(part 1 of 2)
# Autodesk Inventor assembly: gantry_assembly
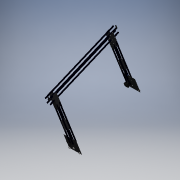
[picture p0: Inventor's stored thumbnail of the model, 180x180]
Saved by Autodesk Inventor 2018 (Build 220112000, 112)
## iProperties
Created: 2017-11-16
Part Number: gantry_assembly
Document SubType Name: Assembly
Designer: g
Author: g
## Documents named in this file (29)
- C:\Users\g\Desktop\AUG_inventor\gantry_assembly.iam
- C:\Users\g\Desktop\AUG_inventor\makerbeam600mm.ipt
- C:\Users\g\Desktop\AUG_inventor\tieplate_small.ipt
- C:\Users\g\Desktop\AUG_inventor\tieplate_big.ipt
- C:\Users\g\Desktop\AUG_inventor\M3 X 10mm Screw.ipt
- C:\Users\g\Desktop\AUG_inventor\M3_Lock_Nut(Thin_Nut).ipt
- C:\Users\g\Desktop\AUG_inventor\tieplate_small_MIR2.ipt
- C:\Users\g\Desktop\AUG_inventor\makerbeam876mm.ipt
- C:\Users\g\Desktop\AUG_inventor\makerbeam600mm_MIR.ipt
- C:\Users\g\Desktop\AUG_inventor\tieplate_small_MIR3.ipt
- C:\Users\g\Desktop\AUG_inventor\tieplate_big_MIR.ipt
- C:\Users\g\Desktop\AUG_inventor\M3 X 10mm Screw_MIR5.ipt
- C:\Users\g\Desktop\AUG_inventor\M3_Lock_Nut(Thin_Nut)_MIR8.ipt
- C:\Users\g\Desktop\AUG_inventor\tieplate_small_MIR2_MIR.ipt
- C:\Users\g\Desktop\AUG_inventor\NEMA17 w connector metric.ipt
- C:\Users\g\Desktop\AUG_inventor\GT2Pulley metric.ipt
- C:\Users\g\Desktop\AUG_inventor\GT2Bearing metric.ipt
- C:\Users\g\Desktop\AUG_inventor\M5 x 12mm Screw.ipt
- C:\Users\g\Desktop\AUG_inventor\M5 x 12mm Screw_MIR.ipt
- C:\Users\g\Desktop\AUG_inventor\m5x12mmscrew.ipt
- C:\Users\g\Desktop\AUG_inventor\5mmx20mmx8mm bearing.ipt
- C:\Users\g\Desktop\AUG_inventor\NEMA17 w connector metric_MIR.ipt
- C:\Users\g\Desktop\AUG_inventor\GT2Pulley metric_MIR.ipt
- C:\Users\g\Desktop\AUG_inventor\GT2Bearing metric_MIR.ipt
- C:\Users\g\Desktop\AUG_inventor\M5 x 12mm Screw_MIR1.ipt
- C:\Users\g\Desktop\AUG_inventor\M5 x 12mm Screw_MIR_MIR.ipt
- C:\Users\g\Desktop\AUG_inventor\m5x12mmscrew_MIR.ipt
- C:\Users\g\Desktop\AUG_inventor\5mmx20mmx8mm bearing_MIR.ipt
- C:\Users\g\Desktop\AUG_inventor\makerbeam_L-bracket.ipt
## Components (276 placed, 28 different names)
1. makerbeam600mm:1 — Mate:3, Flush:8, Flush:9, Mate:10, Flush:13, Flush:14, Mate:16, Slider:1, Slider:2, Flush:22, Slider:3, Flush:23, Slider:13, Slider:18, Slider:21, Slider:28, Slider:29, Slider:30, Flush:127, Flush:132, Flush:147, Flush:148
2. makerbeam600mm:2 — Mate:9, Flush:11, Mate:13, Flush:19, Flush:20, Mate:17, Mate:18, Flush:31, Flush:32, Mate:40, Slider:7, Flush:33, Slider:8, Slider:9, Flush:34, Slider:14, Slider:17, Slider:22, Slider:25, Slider:26, Slider:27, Slider:39, Slider:40, Mate:95, Flush:128, Flush:133, Flush:149, Flush:150
3. makerbeam600mm:3 — Mate:5, Flush:16, Mate:15, Flush:18, Flush:30, Mate:41, Slider:10, Slider:11, Slider:12, Slider:16, Slider:19, Slider:24, Slider:31, Slider:32, Slider:33, Slider:37, Slider:38, Mate:97, Flush:130, Flush:134, Flush:151, Flush:152
4. makerbeam600mm:4 — Flush:5, Flush:6, Mate:4, Mate:6, Flush:10, Mate:14, Flush:17, Flush:21, Slider:4, Slider:5, Slider:6, Flush:37, Slider:15, Slider:20, Slider:23, Slider:34, Slider:35, Slider:36, Flush:129, Flush:131
5. tieplate_small:2 — Mate:9, Mate:10, Mate:11, Flush:11, Flush:42, Flush:43, Flush:44, Flush:45, Flush:46, Flush:47, Mate:74, Mate:75, Mate:76, Mate:77, Mate:78, Mate:79
6. tieplate_small:3 — Mate:5, Mate:6, Mate:7, Flush:10, Flush:48, Flush:49, Flush:50, Flush:51, Flush:52, Flush:53, Mate:80, Mate:81, Mate:82, Mate:83, Mate:84, Mate:85
7. tieplate_small:5 — Flush:5, Flush:6, Mate:3, Flush:8, Flush:9, Mate:4, Mate:7, Mate:11, Mate:19, Mate:20, Mate:21, Mate:23, Mate:24, Mate:25, Mate:26, Mate:27, Mate:28, Mate:50, Mate:51, Flush:67, Flush:70, Flush:125, Flush:127, Flush:129, Flush:147, Symmetry:2
8. tieplate_small:6 — Mate:13, Flush:13, Flush:14, Mate:39, Mate:54, Mate:55, Mate:58, Mate:59, Mate:94, Mate:96, Flush:54, Flush:57, Flush:59, Flush:62, Mate:103, Mate:104, Mate:105, Flush:64, Flush:65, Mate:113, Mate:114, Flush:132, Flush:133, Flush:136, Flush:148, Flush:150
9. tieplate_small:7 — Mate:14, Flush:16, Mate:56, Mate:57, Mate:60, Mate:61, Mate:98, Mate:99, Flush:55, Flush:56, Flush:58, Flush:60, Mate:100, Mate:108, Mate:109, Flush:66, Mate:112, Mate:115, Mate:116, Mate:117, Flush:131, Flush:134, Flush:135, Flush:152
10. tieplate_small:8 — Mate:15, Flush:17, Flush:18, Mate:38, Mate:50, Mate:52, Flush:37, Flush:40, Flush:41, Mate:62, Mate:63, Mate:66, Mate:68, Mate:69, Mate:70, Flush:63, Mate:101, Mate:106, Mate:107, Flush:138
11. tieplate_small:9 — Mate:16, Flush:19, Flush:20, Mate:51, Mate:53, Flush:38, Flush:39, Mate:64, Mate:65, Mate:67, Mate:71, Mate:72, Mate:73, Flush:61, Mate:102, Mate:110, Mate:111, Flush:137
12. tieplate_big:1 — Mate:17, Mate:18, Flush:21, Mate:86, Mate:87, Mate:88, Mate:89, Mate:90, Mate:91, Mate:92, Mate:93, Mate:226, Flush:161, Flush:162, Mate:227, Flush:163, Mate:228, Flush:164, Mate:232, Mate:233, Mate:239, Mate:240, Mate:241, Mate:244, Cylindrical:107, Mate:245, Mate:246, Cylindrical:108, Cylindrical:109
13. M3 X 10mm Screw:1 — Cylindrical:9, Mate:44
14. M3 X 10mm Screw:2 — Cylindrical:10, Mate:45
15. M3 X 10mm Screw:3 — Cylindrical:11, Mate:48
16. M3 X 10mm Screw:4 — Cylindrical:2, Mate:25
17. M3 X 10mm Screw:5 — Cylindrical:1, Mate:24
18. M3 X 10mm Screw:6 — Cylindrical:5, Mate:26
19. M3 X 10mm Screw:7 — Cylindrical:6, Mate:27
20. M3 X 10mm Screw:8 — Cylindrical:7, Mate:47
21. M3 X 10mm Screw:9 — Cylindrical:16, Mate:60
22. M3 X 10mm Screw:10 — Cylindrical:17, Mate:59
23. M3 X 10mm Screw:11 — Cylindrical:15, Mate:61
24. M3 X 10mm Screw:12 — Cylindrical:14, Mate:49
25. M3 X 10mm Screw:13 — Cylindrical:4, Mate:23
26. M3 X 10mm Screw:14 — Cylindrical:3, Mate:28
27. M3 X 10mm Screw:15 — Cylindrical:8, Mate:46
28. M3_Lock_Nut(Thin_Nut):2 — Slider:20, Flush:41, Cylindrical:22
29. M3_Lock_Nut(Thin_Nut):3 — Slider:19, Flush:40, Cylindrical:21
30. M3_Lock_Nut(Thin_Nut):4 — Slider:18, Flush:39, Cylindrical:19
31. M3_Lock_Nut(Thin_Nut):5 — Slider:2, Flush:22, Cylindrical:2, Flush:25
32. M3_Lock_Nut(Thin_Nut):6 — Slider:1, Mate:19, Cylindrical:3, Flush:24
33. M3_Lock_Nut(Thin_Nut):7 — Slider:14, Mate:54, Cylindrical:18
34. M3_Lock_Nut(Thin_Nut):8 — Slider:17, Flush:38, Cylindrical:20
35. M3_Lock_Nut(Thin_Nut):9 — Slider:4, Flush:24, Cylindrical:6
36. M3_Lock_Nut(Thin_Nut):10 — Slider:5, Flush:25, Cylindrical:5
37. M3_Lock_Nut(Thin_Nut):11 — Slider:22, Mate:65, Cylindrical:23
38. M3_Lock_Nut(Thin_Nut):12 — Slider:13, Mate:55, Cylindrical:17
39. M3_Lock_Nut(Thin_Nut):13 — Slider:3, Flush:23, Cylindrical:1, Flush:26
40. M3_Lock_Nut(Thin_Nut):14 — Slider:6, Flush:26, Cylindrical:4
41. M3_Lock_Nut(Thin_Nut):15 — Slider:15, Mate:57, Cylindrical:15
42. M3_Lock_Nut(Thin_Nut):16 — Slider:16, Mate:56, Cylindrical:16
43. tieplate_small_MIR2:1 — Mate:36, Mate:37, Mate:38, Mate:39, Flush:30, Flush:31, Flush:32, Mate:40, Mate:41, Mate:42, Flush:35, Flush:36, Mate:43, Mate:44, Mate:45, Mate:46, Mate:47, Mate:48, Mate:49, Mate:52, Mate:53, Flush:68, Flush:69, Flush:126, Flush:128, Flush:130, Flush:149, Flush:151
44. M3_Lock_Nut(Thin_Nut):17 — Slider:10, Flush:35, Cylindrical:10
45. M3_Lock_Nut(Thin_Nut):18 — Slider:9, Flush:34, Cylindrical:8
46. M3_Lock_Nut(Thin_Nut):19 — Slider:12, Mate:43, Cylindrical:11
47. M3_Lock_Nut(Thin_Nut):20 — Slider:11, Flush:36, Cylindrical:14
48. M3_Lock_Nut(Thin_Nut):21 — Slider:8, Mate:42, Cylindrical:7
49. M3_Lock_Nut(Thin_Nut):22 — Slider:7, Flush:33, Cylindrical:9
50. M3 X 10mm Screw:16 — Cylindrical:18, Mate:58
51. M3_Lock_Nut(Thin_Nut):23 — Slider:24, Mate:62, Cylindrical:26
52. M3_Lock_Nut(Thin_Nut):24 — Slider:23, Mate:63, Cylindrical:25
53. M3_Lock_Nut(Thin_Nut):25 — Slider:21, Mate:64, Cylindrical:24
54. M3 X 10mm Screw:17 — Cylindrical:19, Mate:72
55. M3 X 10mm Screw:18 — Cylindrical:20, Mate:73
56. M3 X 10mm Screw:19 — Cylindrical:21, Mate:68
57. M3 X 10mm Screw:20 — Cylindrical:22, Mate:70
58. M3 X 10mm Screw:21 — Cylindrical:26, Mate:66
59. M3 X 10mm Screw:22 — Cylindrical:25, Mate:69
60. M3 X 10mm Screw:23 — Cylindrical:24, Mate:71
61. M3 X 10mm Screw:24 — Cylindrical:23, Mate:67
62. M3 X 10mm Screw:25 — Cylindrical:33, Mate:74
63. M3 X 10mm Screw:26 — Cylindrical:37, Mate:79
64. M3 X 10mm Screw:27 — Cylindrical:31, Mate:82
65. M3 X 10mm Screw:28 — Cylindrical:34, Mate:75
66. M3 X 10mm Screw:29 — Cylindrical:36, Mate:78
67. M3 X 10mm Screw:30 — Cylindrical:29, Mate:81
68. M3 X 10mm Screw:31 — Cylindrical:38, Mate:77
69. M3 X 10mm Screw:32 — Cylindrical:32, Mate:85
70. M3 X 10mm Screw:33 — Cylindrical:28, Mate:83
71. M3 X 10mm Screw:34 — Cylindrical:35, Mate:76
72. M3 X 10mm Screw:35 — Cylindrical:30, Mate:80
73. M3 X 10mm Screw:36 — Cylindrical:27, Mate:84
74. M3_Lock_Nut(Thin_Nut):26 — Slider:25, Flush:42, Cylindrical:37
75. M3_Lock_Nut(Thin_Nut):27 — Slider:26, Flush:44, Cylindrical:38
76. M3_Lock_Nut(Thin_Nut):28 — Slider:28, Flush:46, Cylindrical:34
77. M3_Lock_Nut(Thin_Nut):29 — Slider:27, Flush:43, Cylindrical:36
78. M3_Lock_Nut(Thin_Nut):30 — Slider:34, Flush:50, Cylindrical:27
79. M3_Lock_Nut(Thin_Nut):31 — Slider:32, Flush:53, Cylindrical:32
80. M3_Lock_Nut(Thin_Nut):32 — Slider:29, Flush:45, Cylindrical:33
81. M3_Lock_Nut(Thin_Nut):33 — Slider:33, Flush:51, Cylindrical:30
82. M3_Lock_Nut(Thin_Nut):34 — Slider:36, Flush:49, Cylindrical:28
83. M3_Lock_Nut(Thin_Nut):35 — Slider:30, Flush:47, Cylindrical:35
84. M3_Lock_Nut(Thin_Nut):36 — Slider:31, Flush:52, Cylindrical:31
85. M3_Lock_Nut(Thin_Nut):37 — Slider:35, Flush:48, Cylindrical:29
86. M3_Lock_Nut(Thin_Nut):39 — Slider:37, Mate:86, Cylindrical:42
87. M3_Lock_Nut(Thin_Nut):40 — Slider:38, Mate:87, Cylindrical:39
88. M3_Lock_Nut(Thin_Nut):41 — Slider:40, Mate:88, Cylindrical:41
89. M3_Lock_Nut(Thin_Nut):42 — Slider:39, Mate:89, Cylindrical:40
90. M3 X 10mm Screw:37 — Cylindrical:39, Mate:91
91. M3 X 10mm Screw:38 — Cylindrical:42, Mate:90
92. M3 X 10mm Screw:39 — Cylindrical:40, Mate:92
93. M3 X 10mm Screw:40 — Cylindrical:41, Mate:93
94. makerbeam876mm:1 — Mate:96, Flush:54, Flush:57, Slider:51, Slider:52, Flush:136, Flush:140, Slider:95, Slider:101, Flush:189, Flush:190, Flush:192
95. makerbeam876mm:2 — Mate:94, Mate:95, Flush:59, Slider:43, Slider:44, Slider:45, Slider:46, Flush:69, Flush:70, Flush:125, Flush:126, Flush:137, Flush:141, Slider:93, Slider:94, Slider:104, Slider:105, Flush:188, Flush:189
96. makerbeam876mm:3 — Mate:99, Flush:55, Flush:56, Slider:49, Slider:50, Symmetry:1, Flush:135, Flush:139, Slider:99, Slider:100, Flush:182, Mate:320, Flush:183, Flush:184, Flush:185, Mate:321, Slider:106, Slider:107, Flush:186, Slider:108, Slider:109, Flush:190, Flush:191
97. makerbeam876mm:4 — Mate:97, Mate:98, Flush:58, Slider:41, Slider:42, Slider:47, Slider:48, Flush:67, Flush:68, Symmetry:1, Flush:123, Flush:124, Flush:138, Flush:142, Slider:97, Slider:98, Slider:102, Slider:103, Flush:160, Flush:188, Flush:191, Flush:192
98. M3_Lock_Nut(Thin_Nut):43 — Slider:43, Mate:103, Cylindrical:49
99. M3_Lock_Nut(Thin_Nut):44 — Slider:42, Mate:101, Cylindrical:47
100. M3_Lock_Nut(Thin_Nut):45 — Slider:41, Flush:63, Cylindrical:48
101. M3_Lock_Nut(Thin_Nut):46 — Slider:44, Flush:62, Cylindrical:50
102. M3_Lock_Nut(Thin_Nut):47 — Slider:45, Flush:61, Cylindrical:45
103. M3_Lock_Nut(Thin_Nut):48 — Slider:46, Mate:102, Cylindrical:46
104. M3_Lock_Nut(Thin_Nut):49 — Slider:47, Flush:60, Cylindrical:44
105. M3_Lock_Nut(Thin_Nut):50 — Slider:48, Mate:100, Cylindrical:43
106. M3_Lock_Nut(Thin_Nut):51 — Slider:50, Flush:66, Cylindrical:51
107. M3_Lock_Nut(Thin_Nut):52 — Slider:52, Flush:65, Cylindrical:54
108. M3_Lock_Nut(Thin_Nut):53 — Slider:49, Mate:112, Cylindrical:52
109. M3_Lock_Nut(Thin_Nut):54 — Slider:51, Flush:64, Cylindrical:53
110. M3 X 10mm Screw:41 — Cylindrical:49, Mate:104
111. M3 X 10mm Screw:42 — Cylindrical:48, Mate:107
112. M3 X 10mm Screw:43 — Cylindrical:50, Mate:105
113. M3 X 10mm Screw:44 — Cylindrical:47, Mate:106
114. M3 X 10mm Screw:45 — Cylindrical:53, Mate:114
115. M3 X 10mm Screw:46 — Cylindrical:51, Mate:115
116. M3 X 10mm Screw:47 — Cylindrical:54, Mate:113
117. M3 X 10mm Screw:48 — Cylindrical:52, Mate:117
118. M3 X 10mm Screw:49 — Cylindrical:46, Mate:110
119. M3 X 10mm Screw:50 — Cylindrical:43, Mate:109, Mate:116
120. M3 X 10mm Screw:51 — Cylindrical:44, Mate:108
121. M3 X 10mm Screw:52 — Cylindrical:45, Mate:111
122. makerbeam600mm_MIR:1 — Mate:118, Flush:75, Flush:76, Mate:125, Flush:79, Flush:80, Mate:131, Flush:91, Flush:95, Slider:55, Slider:56, Slider:57, Slider:63, Slider:64, Slider:76, Slider:79, Slider:83, Slider:86
123. makerbeam600mm_MIR:2 — Flush:73, Mate:119, Mate:126, Flush:85, Flush:86, Mate:132, Mate:133, Mate:160, Flush:97, Flush:98, Flush:101, Flush:103, Slider:58, Slider:59, Slider:62, Slider:69, Slider:72, Slider:73, Slider:77, Slider:78, Slider:80, Slider:91, Slider:92
124. makerbeam600mm_MIR:3 — Mate:121, Flush:81, Flush:83, Mate:129, Mate:159, Flush:99, Slider:54, Slider:67, Slider:68, Slider:70, Slider:71, Slider:74, Slider:82, Slider:84, Slider:87, Slider:89, Slider:90, Flush:145, Flush:146
125. makerbeam600mm_MIR:4 — Flush:74, Mate:120, Mate:124, Flush:77, Flush:78, Mate:127, Flush:82, Flush:84, Flush:87, Slider:53, Slider:60, Slider:61, Slider:65, Slider:66, Slider:75, Slider:81, Slider:85, Slider:88, Flush:143, Flush:144
126. tieplate_small_MIR3:1 — Flush:73, Mate:118, Mate:119, Mate:122, Mate:179, Mate:180, Mate:182, Mate:183, Mate:185, Mate:188, Flush:104, Flush:105, Flush:106, Flush:107, Flush:110, Flush:113
127. tieplate_small_MIR3:2 — Flush:74, Mate:120, Mate:121, Mate:123, Mate:181, Mate:184, Mate:186, Mate:187, Mate:189, Mate:190, Flush:108, Flush:109, Flush:111, Flush:112, Flush:114, Flush:115
128. tieplate_small_MIR3:3 — Mate:122, Mate:123, Mate:124, Flush:75, Flush:76, Mate:125, Flush:77, Flush:78, Mate:128, Mate:130, Mate:134, Mate:135, Mate:136, Mate:137, Mate:141, Mate:142, Mate:143, Mate:149, Mate:150, Flush:123, Flush:143, Symmetry:2
129. tieplate_small_MIR3:4 — Flush:79, Flush:80, Mate:126, Mate:139, Mate:144, Mate:146, Mate:161, Mate:167, Mate:199, Flush:117, Flush:121, Mate:204, Mate:206, Mate:210, Flush:140, Flush:155, Mate:218, Mate:219, Mate:224, Mate:225
130. tieplate_small_MIR3:5 — Flush:81, Mate:127, Mate:138, Mate:140, Mate:147, Mate:148, Flush:119, Mate:202, Mate:209, Mate:211, Mate:213, Mate:214, Mate:215, Flush:139, Flush:144, Flush:146, Flush:153, Mate:217, Flush:154, Mate:220, Mate:221, Mate:222, Mate:223, Flush:160
131. tieplate_small_MIR3:6 — Flush:82, Mate:128, Flush:83, Flush:84, Mate:129, Flush:88, Flush:89, Mate:152, Mate:162, Mate:168, Mate:169, Mate:173, Mate:174, Mate:175, Mate:176, Mate:200, Flush:116, Mate:205, Mate:207, Flush:142
132. tieplate_small_MIR3:7 — Mate:130, Flush:85, Flush:86, Mate:131, Flush:90, Flush:92, Mate:145, Mate:151, Mate:170, Mate:171, Mate:172, Mate:177, Mate:178, Flush:118, Mate:201, Mate:212, Mate:216, Flush:141
133. tieplate_big_MIR:1 — Flush:87, Mate:132, Mate:133, Mate:191, Mate:192, Mate:193, Mate:194, Mate:195, Mate:196, Mate:197, Mate:198, Mate:250, Mate:251, Mate:252, Mate:253, Mate:255, Mate:256, Cylindrical:110, Cylindrical:111, Cylindrical:112, Mate:257, Flush:165, Mate:258, Mate:259, Mate:302, Mate:303, Mate:304
134. M3 X 10mm Screw_MIR5:1 — Mate:158, Cylindrical:69
135. M3 X 10mm Screw_MIR5:2 — Mate:157, Cylindrical:64
136. M3 X 10mm Screw_MIR5:3 — Mate:154, Cylindrical:66
137. M3 X 10mm Screw_MIR5:4 — Mate:134, Cylindrical:55
138. M3 X 10mm Screw_MIR5:5 — Mate:135, Cylindrical:60
139. M3 X 10mm Screw_MIR5:6 — Mate:136, Cylindrical:58
140. M3 X 10mm Screw_MIR5:7 — Mate:137, Cylindrical:57
141. M3 X 10mm Screw_MIR5:8 — Mate:155, Cylindrical:68
142. M3 X 10mm Screw_MIR5:9 — Mate:138, Cylindrical:63
143. M3 X 10mm Screw_MIR5:10 — Mate:139, Cylindrical:59
144. M3 X 10mm Screw_MIR5:11 — Mate:140, Cylindrical:62
145. M3 X 10mm Screw_MIR5:12 — Mate:153, Cylindrical:67
146. M3 X 10mm Screw_MIR5:13 — Mate:141, Cylindrical:61
147. M3 X 10mm Screw_MIR5:14 — Mate:142, Cylindrical:56
148. M3 X 10mm Screw_MIR5:15 — Mate:156, Cylindrical:65
149. M3_Lock_Nut(Thin_Nut)_MIR8:1 — Flush:88, Slider:53, Cylindrical:74
150. M3_Lock_Nut(Thin_Nut)_MIR8:2 — Flush:89, Slider:54, Cylindrical:73
151. M3_Lock_Nut(Thin_Nut)_MIR8:3 — Flush:90, Slider:55, Cylindrical:71
152. M3_Lock_Nut(Thin_Nut)_MIR8:4 — Flush:91, Flush:94, Cylindrical:55, Slider:56
153. M3_Lock_Nut(Thin_Nut)_MIR8:5 — Mate:143, Flush:93, Cylindrical:56, Slider:57
154. M3_Lock_Nut(Thin_Nut)_MIR8:6 — Mate:144, Slider:58, Cylindrical:70
155. M3_Lock_Nut(Thin_Nut)_MIR8:7 — Flush:92, Slider:59, Cylindrical:72
156. M3_Lock_Nut(Thin_Nut)_MIR8:8 — Flush:93, Cylindrical:57, Slider:60
157. M3_Lock_Nut(Thin_Nut)_MIR8:9 — Flush:94, Cylindrical:58, Slider:61
158. M3_Lock_Nut(Thin_Nut)_MIR8:10 — Mate:145, Slider:62, Cylindrical:78
159. M3_Lock_Nut(Thin_Nut)_MIR8:11 — Mate:146, Cylindrical:59, Slider:63
160. M3_Lock_Nut(Thin_Nut)_MIR8:12 — Flush:95, Flush:96, Cylindrical:60, Slider:64
161. M3_Lock_Nut(Thin_Nut)_MIR8:13 — Flush:96, Cylindrical:61, Slider:65
162. M3_Lock_Nut(Thin_Nut)_MIR8:14 — Mate:147, Cylindrical:62, Slider:66
163. M3_Lock_Nut(Thin_Nut)_MIR8:15 — Mate:148, Cylindrical:63, Slider:67
164. tieplate_small_MIR2_MIR:1 — Mate:151, Mate:152, Mate:153, Mate:154, Mate:155, Mate:156, Mate:157, Mate:158, Mate:159, Mate:160, Flush:97, Flush:98, Flush:99, Mate:161, Mate:162, Mate:163, Mate:164, Flush:100, Mate:165, Flush:102, Mate:166, Flush:124, Flush:145
165. M3_Lock_Nut(Thin_Nut)_MIR8:16 — Flush:100, Cylindrical:64, Slider:68
166. M3_Lock_Nut(Thin_Nut)_MIR8:17 — Flush:101, Cylindrical:65, Slider:69
167. M3_Lock_Nut(Thin_Nut)_MIR8:18 — Mate:165, Cylindrical:66, Slider:70
168. M3_Lock_Nut(Thin_Nut)_MIR8:19 — Flush:102, Cylindrical:67, Slider:71
169. M3_Lock_Nut(Thin_Nut)_MIR8:20 — Mate:166, Cylindrical:68, Slider:72
170. M3_Lock_Nut(Thin_Nut)_MIR8:21 — Flush:103, Cylindrical:69, Slider:73
171. M3 X 10mm Screw_MIR5:16 — Mate:167, Cylindrical:70
172. M3_Lock_Nut(Thin_Nut)_MIR8:22 — Mate:168, Slider:74, Cylindrical:75
173. M3_Lock_Nut(Thin_Nut)_MIR8:23 — Mate:169, Slider:75, Cylindrical:76
174. M3_Lock_Nut(Thin_Nut)_MIR8:24 — Mate:170, Slider:76, Cylindrical:77
175. M3 X 10mm Screw_MIR5:17 — Mate:171, Cylindrical:71
176. M3 X 10mm Screw_MIR5:18 — Mate:172, Cylindrical:72
177. M3 X 10mm Screw_MIR5:19 — Mate:173, Cylindrical:73
178. M3 X 10mm Screw_MIR5:20 — Mate:174, Cylindrical:74
179. M3 X 10mm Screw_MIR5:21 — Mate:175, Cylindrical:75
180. M3 X 10mm Screw_MIR5:22 — Mate:176, Cylindrical:76
181. M3 X 10mm Screw_MIR5:23 — Mate:177, Cylindrical:77
182. M3 X 10mm Screw_MIR5:24 — Mate:178, Cylindrical:78
183. M3 X 10mm Screw_MIR5:25 — Mate:179, Cylindrical:85
184. M3 X 10mm Screw_MIR5:26 — Mate:180, Cylindrical:79
185. M3 X 10mm Screw_MIR5:27 — Mate:181, Cylindrical:89
186. M3 X 10mm Screw_MIR5:28 — Mate:182, Cylindrical:81
187. M3 X 10mm Screw_MIR5:29 — Mate:183, Cylindrical:82
188. M3 X 10mm Screw_MIR5:30 — Mate:184, Cylindrical:90
189. M3 X 10mm Screw_MIR5:31 — Mate:185, Cylindrical:80
190. M3 X 10mm Screw_MIR5:32 — Mate:186, Cylindrical:84
191. M3 X 10mm Screw_MIR5:33 — Mate:187, Cylindrical:87
192. M3 X 10mm Screw_MIR5:34 — Mate:188, Cylindrical:88
193. M3 X 10mm Screw_MIR5:35 — Mate:189, Cylindrical:86
194. M3 X 10mm Screw_MIR5:36 — Mate:190, Cylindrical:83
195. M3_Lock_Nut(Thin_Nut)_MIR8:25 — Flush:104, Cylindrical:79, Slider:77
196. M3_Lock_Nut(Thin_Nut)_MIR8:26 — Flush:105, Cylindrical:80, Slider:78
197. M3_Lock_Nut(Thin_Nut)_MIR8:27 — Flush:106, Cylindrical:81, Slider:79
198. M3_Lock_Nut(Thin_Nut)_MIR8:28 — Flush:107, Cylindrical:82, Slider:80
199. M3_Lock_Nut(Thin_Nut)_MIR8:29 — Flush:108, Cylindrical:83, Slider:81
200. M3_Lock_Nut(Thin_Nut)_MIR8:30 — Flush:109, Cylindrical:84, Slider:82
201. M3_Lock_Nut(Thin_Nut)_MIR8:31 — Flush:110, Cylindrical:85, Slider:83
202. M3_Lock_Nut(Thin_Nut)_MIR8:32 — Flush:111, Cylindrical:86, Slider:84
203. M3_Lock_Nut(Thin_Nut)_MIR8:33 — Flush:112, Cylindrical:87, Slider:85
204. M3_Lock_Nut(Thin_Nut)_MIR8:34 — Flush:113, Cylindrical:88, Slider:86
205. M3_Lock_Nut(Thin_Nut)_MIR8:35 — Flush:114, Cylindrical:89, Slider:87
206. M3_Lock_Nut(Thin_Nut)_MIR8:36 — Flush:115, Cylindrical:90, Slider:88
207. M3_Lock_Nut(Thin_Nut)_MIR8:37 — Mate:191, Slider:89, Cylindrical:92
208. M3_Lock_Nut(Thin_Nut)_MIR8:38 — Mate:192, Slider:90, Cylindrical:91
209. M3_Lock_Nut(Thin_Nut)_MIR8:39 — Mate:193, Slider:91, Cylindrical:94
210. M3_Lock_Nut(Thin_Nut)_MIR8:40 — Mate:194, Slider:92, Cylindrical:93
211. M3 X 10mm Screw_MIR5:37 — Mate:195, Cylindrical:91
212. M3 X 10mm Screw_MIR5:38 — Mate:196, Cylindrical:92
213. M3 X 10mm Screw_MIR5:39 — Mate:197, Cylindrical:93
214. M3 X 10mm Screw_MIR5:40 — Mate:198, Cylindrical:94
215. M3_Lock_Nut(Thin_Nut)_MIR8:41 — Mate:199, Cylindrical:95, Slider:94
216. M3_Lock_Nut(Thin_Nut)_MIR8:42 — Mate:200, Cylindrical:98, Slider:103
217. M3_Lock_Nut(Thin_Nut)_MIR8:43 — Flush:116, Cylindrical:96, Slider:102
218. M3_Lock_Nut(Thin_Nut)_MIR8:44 — Flush:117, Cylindrical:97, Slider:93
219. M3_Lock_Nut(Thin_Nut)_MIR8:45 — Flush:118, Cylindrical:106, Slider:105
220. M3_Lock_Nut(Thin_Nut)_MIR8:46 — Mate:201, Cylindrical:103, Slider:104
221. M3_Lock_Nut(Thin_Nut)_MIR8:47 — Flush:119, Cylindrical:105, Slider:97, Flush:154
222. M3_Lock_Nut(Thin_Nut)_MIR8:48 — Mate:202, Cylindrical:104, Slider:98
223. M3_Lock_Nut(Thin_Nut)_MIR8:49 — Cylindrical:100, Slider:99, Mate:217
224. M3_Lock_Nut(Thin_Nut)_MIR8:50 — Flush:121, Cylindrical:101, Slider:95
225. M3_Lock_Nut(Thin_Nut)_MIR8:51 — Cylindrical:102, Slider:100, Flush:153
226. M3_Lock_Nut(Thin_Nut)_MIR8:52 — Cylindrical:99, Slider:101, Flush:155
227. M3 X 10mm Screw_MIR5:41 — Mate:204, Cylindrical:95, Mate:224
228. M3 X 10mm Screw_MIR5:42 — Mate:205, Cylindrical:96
229. M3 X 10mm Screw_MIR5:43 — Mate:206, Cylindrical:97, Mate:225
230. M3 X 10mm Screw_MIR5:44 — Mate:207, Cylindrical:98
231. M3 X 10mm Screw_MIR5:45 — Cylindrical:99, Mate:218
232. M3 X 10mm Screw_MIR5:46 — Mate:209, Cylindrical:100, Mate:221
233. M3 X 10mm Screw_MIR5:47 — Mate:210, Cylindrical:101, Mate:219
234. M3 X 10mm Screw_MIR5:48 — Mate:211, Cylindrical:102, Mate:220
235. M3 X 10mm Screw_MIR5:49 — Mate:212, Cylindrical:103
236. M3 X 10mm Screw_MIR5:50 — Mate:213, Mate:214, Cylindrical:104, Mate:223
237. M3 X 10mm Screw_MIR5:51 — Mate:215, Cylindrical:105, Mate:222
238. M3 X 10mm Screw_MIR5:52 — Mate:216, Cylindrical:106
239. NEMA17 w connector metric:3 — Mate:226, Flush:161, Flush:162, Mate:229, Mate:230, Mate:231, Rigid:3
240. GT2Pulley metric:1 — Rigid:3
241. GT2Bearing metric:3 — Rigid:4
242. GT2Bearing metric:4 — Rigid:2
243. M5 x 12mm Screw:1 — Mate:227, Flush:163, Mate:228, Rigid:2
244. M5 x 12mm Screw_MIR:1 — Flush:164, Mate:232, Mate:233, Rigid:4
245. m5x12mmscrew:1 — Mate:244, Cylindrical:107, Rotational:2
246. m5x12mmscrew:2 — Mate:245, Cylindrical:109, Rotational:1
247. m5x12mmscrew:3 — Mate:246, Cylindrical:108, Rotational:3
248. 5mmx20mmx8mm bearing:1 — Rotational:1
249. 5mmx20mmx8mm bearing:2 — Rotational:2
250. 5mmx20mmx8mm bearing:3 — Rotational:3
251. NEMA17 w connector metric_MIR:1 — Mate:247, Mate:248, Mate:249, Rigid:5, Mate:252, Mate:257, Flush:165
252. GT2Pulley metric_MIR:1 — Rigid:5
253. GT2Bearing metric_MIR:1 — Rigid:7
254. GT2Bearing metric_MIR:2 — Rigid:6
255. M5 x 12mm Screw_MIR1:1 — Rigid:6, Mate:253, Flush:166, Mate:303, Mate:304
256. M5 x 12mm Screw_MIR_MIR:1 — Rigid:7, Mate:258, Mate:259, Flush:166, Mate:302
257. m5x12mmscrew_MIR:1 — Rotational:5, Mate:251, Mate:256, Cylindrical:112
258. m5x12mmscrew_MIR:2 — Rotational:4, Mate:250, Cylindrical:110
259. m5x12mmscrew_MIR:3 — Rotational:6, Mate:255, Cylindrical:111
260. 5mmx20mmx8mm bearing_MIR:1 — Rotational:4
261. 5mmx20mmx8mm bearing_MIR:2 — Rotational:5
262. 5mmx20mmx8mm bearing_MIR:3 — Rotational:6
263. makerbeam_L-bracket:1 — Flush:182, Mate:320, Flush:183, Flush:187, Mate:323, Mate:325, Mate:326, Cylindrical:137, Mate:328, Mate:330
264. makerbeam_L-bracket:2 — Flush:184, Flush:185, Mate:321, Mate:322, Mate:324, Mate:327, Cylindrical:136, Mate:329, Mate:331
265. M3_Lock_Nut(Thin_Nut):55 — Slider:106, Mate:322, Cylindrical:135
266. M3_Lock_Nut(Thin_Nut):56 — Slider:107, Flush:186, Cylindrical:134
267. M3_Lock_Nut(Thin_Nut):57 — Slider:108, Mate:323, Cylindrical:132
268. M3_Lock_Nut(Thin_Nut):58 — Slider:109, Flush:187, Cylindrical:133
269. M3 X 10mm Screw:61 — Cylindrical:132, Mate:325
270. M3 X 10mm Screw:62 — Cylindrical:133, Mate:326
271. M3 X 10mm Screw:63 — Cylindrical:134, Mate:324
272. M3 X 10mm Screw:64 — Cylindrical:135, Mate:327
273. M3 X 10mm Screw:65 — Cylindrical:136, Mate:329, Cylindrical:138
274. M3 X 10mm Screw:66 — Cylindrical:137, Mate:328, Cylindrical:139
275. M3_Lock_Nut(Thin_Nut):59 — Cylindrical:138, Mate:331
276. M3_Lock_Nut(Thin_Nut):60 — Cylindrical:139, Mate:330
## Relationships (651: Mate 252, Flush 159, CylindricalJoint 118, TranslationJoint 108, WeldJoint 6, RevoluteJoint 6, Symmetry 2)
- Flush:5: makerbeam600mm:4 ↔ tieplate_small:5
- Flush:6: makerbeam600mm:4 ↔ tieplate_small:5
- Mate:3: makerbeam600mm:1 ↔ tieplate_small:5
- Flush:8: makerbeam600mm:1 ↔ tieplate_small:5
- Flush:9: makerbeam600mm:1 ↔ tieplate_small:5
- Mate:4: makerbeam600mm:4 ↔ tieplate_small:5
- Mate:5: makerbeam600mm:3 ↔ tieplate_small:3
- Mate:6: makerbeam600mm:4 ↔ tieplate_small:3
- Mate:7: tieplate_small:3 ↔ tieplate_small:5
- Flush:10 (300 mm): makerbeam600mm:4 ↔ tieplate_small:3
- Mate:9: makerbeam600mm:2 ↔ tieplate_small:2
- Mate:10: makerbeam600mm:1 ↔ tieplate_small:2
- Mate:11: tieplate_small:2 ↔ tieplate_small:5
- Flush:11 (300 mm): makerbeam600mm:2 ↔ tieplate_small:2
- Mate:13: makerbeam600mm:2 ↔ tieplate_small:6
- Flush:13: makerbeam600mm:1 ↔ tieplate_small:6
- Flush:14 (-72.5 mm): makerbeam600mm:1 ↔ tieplate_small:6
- Mate:14: makerbeam600mm:4 ↔ tieplate_small:7
- Flush:16 (-72.5 mm): makerbeam600mm:3 ↔ tieplate_small:7
- Mate:15: makerbeam600mm:3 ↔ tieplate_small:8
- Flush:17: makerbeam600mm:4 ↔ tieplate_small:8
- Flush:18 (-10 mm): makerbeam600mm:3 ↔ tieplate_small:8
- Mate:16: makerbeam600mm:1 ↔ tieplate_small:9
- Flush:19: makerbeam600mm:2 ↔ tieplate_small:9
- Flush:20 (-10 mm): makerbeam600mm:2 ↔ tieplate_small:9
- Mate:17: makerbeam600mm:2 ↔ tieplate_big:1
- Mate:18 (-70 mm): makerbeam600mm:2 ↔ tieplate_big:1
- Flush:21 (-50 mm): makerbeam600mm:4 ↔ tieplate_big:1
- Slider:1 [TranslationJoint]: makerbeam600mm:1 ↔ M3_Lock_Nut(Thin_Nut):6
- Mate:19 (-10.5 mm): tieplate_small:5 ↔ M3_Lock_Nut(Thin_Nut):6
- Slider:2 [TranslationJoint]: makerbeam600mm:1 ↔ M3_Lock_Nut(Thin_Nut):5
- Flush:22 (62.5 mm): makerbeam600mm:1 ↔ M3_Lock_Nut(Thin_Nut):5
- Slider:3 [TranslationJoint]: makerbeam600mm:1 ↔ M3_Lock_Nut(Thin_Nut):13
- Flush:23 (5 mm): makerbeam600mm:1 ↔ M3_Lock_Nut(Thin_Nut):13
- Mate:20: tieplate_small:5
- Mate:21: tieplate_small:5
- Cylindrical:1: M3 X 10mm Screw:5 ↔ M3_Lock_Nut(Thin_Nut):13
- Cylindrical:2: M3 X 10mm Screw:4 ↔ M3_Lock_Nut(Thin_Nut):5
- Cylindrical:3: M3 X 10mm Screw:14 ↔ M3_Lock_Nut(Thin_Nut):6
- Slider:4 [TranslationJoint]: makerbeam600mm:4 ↔ M3_Lock_Nut(Thin_Nut):9
- Flush:24: M3_Lock_Nut(Thin_Nut):6 ↔ M3_Lock_Nut(Thin_Nut):9
- Slider:5 [TranslationJoint]: makerbeam600mm:4 ↔ M3_Lock_Nut(Thin_Nut):10
- Flush:25: M3_Lock_Nut(Thin_Nut):5 ↔ M3_Lock_Nut(Thin_Nut):10
- Slider:6 [TranslationJoint]: makerbeam600mm:4 ↔ M3_Lock_Nut(Thin_Nut):14
- Flush:26: M3_Lock_Nut(Thin_Nut):13 ↔ M3_Lock_Nut(Thin_Nut):14
- Cylindrical:4: M3 X 10mm Screw:13 ↔ M3_Lock_Nut(Thin_Nut):14
- Cylindrical:5: M3 X 10mm Screw:6 ↔ M3_Lock_Nut(Thin_Nut):10
- Cylindrical:6: M3 X 10mm Screw:7 ↔ M3_Lock_Nut(Thin_Nut):9
- Mate:23: tieplate_small:5 ↔ M3 X 10mm Screw:13
- Mate:24: tieplate_small:5 ↔ M3 X 10mm Screw:5
- Mate:25: tieplate_small:5 ↔ M3 X 10mm Screw:4
- Mate:26: tieplate_small:5 ↔ M3 X 10mm Screw:6
- Mate:27: tieplate_small:5 ↔ M3 X 10mm Screw:7
- Mate:28: tieplate_small:5 ↔ M3 X 10mm Screw:14
- Mate:36: tieplate_small_MIR2:1
- Mate:37: tieplate_small_MIR2:1
- Mate:38: tieplate_small:8 ↔ tieplate_small_MIR2:1
- Mate:39: tieplate_small:6 ↔ tieplate_small_MIR2:1
- Flush:30: makerbeam600mm:3 ↔ tieplate_small_MIR2:1
- Flush:31: makerbeam600mm:2 ↔ tieplate_small_MIR2:1
- Flush:32: makerbeam600mm:2 ↔ tieplate_small_MIR2:1
- Mate:40: makerbeam600mm:2 ↔ tieplate_small_MIR2:1
- Mate:41: makerbeam600mm:3 ↔ tieplate_small_MIR2:1
- Slider:7 [TranslationJoint]: makerbeam600mm:2 ↔ M3_Lock_Nut(Thin_Nut):22
- Flush:33 (5 mm): makerbeam600mm:2 ↔ M3_Lock_Nut(Thin_Nut):22
- Slider:8 [TranslationJoint] (2.4 mm): makerbeam600mm:2 ↔ M3_Lock_Nut(Thin_Nut):21
- Mate:42 (-10 mm): tieplate_small_MIR2:1 ↔ M3_Lock_Nut(Thin_Nut):21
- Slider:9 [TranslationJoint] (2.4 mm): makerbeam600mm:2 ↔ M3_Lock_Nut(Thin_Nut):18
- Flush:34 (62.5 mm): makerbeam600mm:2 ↔ M3_Lock_Nut(Thin_Nut):18
- Slider:10 [TranslationJoint] (2.4 mm): makerbeam600mm:3 ↔ M3_Lock_Nut(Thin_Nut):17
- Flush:35 (5 mm): tieplate_small_MIR2:1 ↔ M3_Lock_Nut(Thin_Nut):17
- Slider:11 [TranslationJoint] (2.4 mm): makerbeam600mm:3 ↔ M3_Lock_Nut(Thin_Nut):20
- Flush:36 (62.5 mm): tieplate_small_MIR2:1 ↔ M3_Lock_Nut(Thin_Nut):20
- Slider:12 [TranslationJoint] (2.4 mm): makerbeam600mm:3 ↔ M3_Lock_Nut(Thin_Nut):19
- Mate:43 (-10.5 mm): tieplate_small_MIR2:1 ↔ M3_Lock_Nut(Thin_Nut):19
- Cylindrical:7: M3 X 10mm Screw:8 ↔ M3_Lock_Nut(Thin_Nut):21
- Cylindrical:8: M3 X 10mm Screw:15 ↔ M3_Lock_Nut(Thin_Nut):18
- Cylindrical:9: M3 X 10mm Screw:1 ↔ M3_Lock_Nut(Thin_Nut):22
- Cylindrical:10: M3 X 10mm Screw:2 ↔ M3_Lock_Nut(Thin_Nut):17
- Cylindrical:14: M3 X 10mm Screw:12 ↔ M3_Lock_Nut(Thin_Nut):20
- Cylindrical:11: M3 X 10mm Screw:3 ↔ M3_Lock_Nut(Thin_Nut):19
- Mate:44: M3 X 10mm Screw:1 ↔ tieplate_small_MIR2:1
- Mate:45: M3 X 10mm Screw:2 ↔ tieplate_small_MIR2:1
- Mate:46: M3 X 10mm Screw:15 ↔ tieplate_small_MIR2:1
- Mate:47: M3 X 10mm Screw:8 ↔ tieplate_small_MIR2:1
- Mate:48: M3 X 10mm Screw:3 ↔ tieplate_small_MIR2:1
- Mate:49: M3 X 10mm Screw:12 ↔ tieplate_small_MIR2:1
- Mate:50: tieplate_small:5 ↔ tieplate_small:8
- Mate:51: tieplate_small:5 ↔ tieplate_small:9
- Mate:52: tieplate_small:8 ↔ tieplate_small_MIR2:1
- Mate:53: tieplate_small:9 ↔ tieplate_small_MIR2:1
- Flush:37 (10 mm): makerbeam600mm:4 ↔ tieplate_small:8
- Slider:13 [TranslationJoint]: makerbeam600mm:1 ↔ M3_Lock_Nut(Thin_Nut):12
- Slider:14 [TranslationJoint]: makerbeam600mm:2 ↔ M3_Lock_Nut(Thin_Nut):7
- Mate:54 (-10.5 mm): tieplate_small:6 ↔ M3_Lock_Nut(Thin_Nut):7
- Mate:55 (-10.5 mm): tieplate_small:6 ↔ M3_Lock_Nut(Thin_Nut):12
- Slider:15 [TranslationJoint]: makerbeam600mm:4 ↔ M3_Lock_Nut(Thin_Nut):15
- Slider:16 [TranslationJoint]: makerbeam600mm:3 ↔ M3_Lock_Nut(Thin_Nut):16
- Mate:56 (-10.5 mm): tieplate_small:7 ↔ M3_Lock_Nut(Thin_Nut):16
- Mate:57 (-10.5 mm): tieplate_small:7 ↔ M3_Lock_Nut(Thin_Nut):15
- Cylindrical:15: M3 X 10mm Screw:11 ↔ M3_Lock_Nut(Thin_Nut):15
- Cylindrical:16: M3 X 10mm Screw:9 ↔ M3_Lock_Nut(Thin_Nut):16
- Cylindrical:17: M3 X 10mm Screw:10 ↔ M3_Lock_Nut(Thin_Nut):12
- Cylindrical:18: M3_Lock_Nut(Thin_Nut):7 ↔ M3 X 10mm Screw:16
- Mate:58: tieplate_small:6 ↔ M3 X 10mm Screw:16
- Mate:59: tieplate_small:6 ↔ M3 X 10mm Screw:10
- Mate:60: tieplate_small:7 ↔ M3 X 10mm Screw:9
- Mate:61: tieplate_small:7 ↔ M3 X 10mm Screw:11
- Slider:17 [TranslationJoint]: makerbeam600mm:2 ↔ M3_Lock_Nut(Thin_Nut):8
- Flush:38 (68 mm): tieplate_small:9 ↔ M3_Lock_Nut(Thin_Nut):8
- Slider:18 [TranslationJoint]: makerbeam600mm:1 ↔ M3_Lock_Nut(Thin_Nut):4
- Flush:39 (62.5 mm): tieplate_small:9 ↔ M3_Lock_Nut(Thin_Nut):4
- Slider:19 [TranslationJoint]: makerbeam600mm:3 ↔ M3_Lock_Nut(Thin_Nut):3
- Flush:40 (62.5 mm): tieplate_small:8 ↔ M3_Lock_Nut(Thin_Nut):3
- Slider:20 [TranslationJoint]: makerbeam600mm:4 ↔ M3_Lock_Nut(Thin_Nut):2
- Flush:41 (62.5 mm): tieplate_small:8 ↔ M3_Lock_Nut(Thin_Nut):2
- Slider:21 [TranslationJoint]: makerbeam600mm:1 ↔ M3_Lock_Nut(Thin_Nut):25
- Slider:22 [TranslationJoint]: makerbeam600mm:2 ↔ M3_Lock_Nut(Thin_Nut):11
- Slider:23 [TranslationJoint]: makerbeam600mm:4 ↔ M3_Lock_Nut(Thin_Nut):24
- Slider:24 [TranslationJoint]: makerbeam600mm:3 ↔ M3_Lock_Nut(Thin_Nut):23
- Mate:62 (-10.5 mm): tieplate_small:8 ↔ M3_Lock_Nut(Thin_Nut):23
- Mate:63 (-10.5 mm): tieplate_small:8 ↔ M3_Lock_Nut(Thin_Nut):24
- Mate:64 (-10.5 mm): tieplate_small:9 ↔ M3_Lock_Nut(Thin_Nut):25
- Mate:65 (-10.5 mm): tieplate_small:9 ↔ M3_Lock_Nut(Thin_Nut):11
- Cylindrical:19: M3_Lock_Nut(Thin_Nut):4 ↔ M3 X 10mm Screw:17
- Cylindrical:20: M3_Lock_Nut(Thin_Nut):8 ↔ M3 X 10mm Screw:18
- Cylindrical:21: M3_Lock_Nut(Thin_Nut):3 ↔ M3 X 10mm Screw:19
- Cylindrical:22: M3_Lock_Nut(Thin_Nut):2 ↔ M3 X 10mm Screw:20
- Cylindrical:23: M3_Lock_Nut(Thin_Nut):11 ↔ M3 X 10mm Screw:24
- Cylindrical:24: M3_Lock_Nut(Thin_Nut):25 ↔ M3 X 10mm Screw:23
- Cylindrical:25: M3_Lock_Nut(Thin_Nut):24 ↔ M3 X 10mm Screw:22
- Cylindrical:26: M3_Lock_Nut(Thin_Nut):23 ↔ M3 X 10mm Screw:21
- Mate:66: tieplate_small:8 ↔ M3 X 10mm Screw:21
- Mate:67: tieplate_small:9 ↔ M3 X 10mm Screw:24
- Mate:68: tieplate_small:8 ↔ M3 X 10mm Screw:19
- Mate:69: tieplate_small:8 ↔ M3 X 10mm Screw:22
- Mate:70: tieplate_small:8 ↔ M3 X 10mm Screw:20
- Mate:71: tieplate_small:9 ↔ M3 X 10mm Screw:23
- Mate:72: tieplate_small:9 ↔ M3 X 10mm Screw:17
- Mate:73: tieplate_small:9 ↔ M3 X 10mm Screw:18
- Slider:25 [TranslationJoint]: makerbeam600mm:2 ↔ M3_Lock_Nut(Thin_Nut):26
- Slider:26 [TranslationJoint]: makerbeam600mm:2 ↔ M3_Lock_Nut(Thin_Nut):27
- Slider:27 [TranslationJoint]: makerbeam600mm:2 ↔ M3_Lock_Nut(Thin_Nut):29
- Flush:42 (5 mm): tieplate_small:2 ↔ M3_Lock_Nut(Thin_Nut):26
- Flush:43 (62.5 mm): tieplate_small:2 ↔ M3_Lock_Nut(Thin_Nut):29
- Flush:44 (120 mm): tieplate_small:2 ↔ M3_Lock_Nut(Thin_Nut):27
- Slider:28 [TranslationJoint]: makerbeam600mm:1 ↔ M3_Lock_Nut(Thin_Nut):28
- Slider:29 [TranslationJoint]: makerbeam600mm:1 ↔ M3_Lock_Nut(Thin_Nut):32
- Slider:30 [TranslationJoint]: makerbeam600mm:1 ↔ M3_Lock_Nut(Thin_Nut):35
- Flush:45 (5 mm): tieplate_small:2 ↔ M3_Lock_Nut(Thin_Nut):32
- Flush:46 (62.5 mm): tieplate_small:2 ↔ M3_Lock_Nut(Thin_Nut):28
- Flush:47 (120 mm): tieplate_small:2 ↔ M3_Lock_Nut(Thin_Nut):35
- Slider:31 [TranslationJoint]: makerbeam600mm:3 ↔ M3_Lock_Nut(Thin_Nut):36
- Slider:32 [TranslationJoint]: makerbeam600mm:3 ↔ M3_Lock_Nut(Thin_Nut):31
- Slider:33 [TranslationJoint]: makerbeam600mm:3 ↔ M3_Lock_Nut(Thin_Nut):33
- Slider:34 [TranslationJoint]: makerbeam600mm:4 ↔ M3_Lock_Nut(Thin_Nut):30
- Slider:35 [TranslationJoint]: makerbeam600mm:4 ↔ M3_Lock_Nut(Thin_Nut):37
- Slider:36 [TranslationJoint]: makerbeam600mm:4 ↔ M3_Lock_Nut(Thin_Nut):34
- Flush:48 (5 mm): tieplate_small:3 ↔ M3_Lock_Nut(Thin_Nut):37
- Flush:49 (62.5 mm): tieplate_small:3 ↔ M3_Lock_Nut(Thin_Nut):34
- Flush:50 (120 mm): tieplate_small:3 ↔ M3_Lock_Nut(Thin_Nut):30
- Flush:51 (5 mm): tieplate_small:3 ↔ M3_Lock_Nut(Thin_Nut):33
- Flush:52 (62.5 mm): tieplate_small:3 ↔ M3_Lock_Nut(Thin_Nut):36
- Flush:53 (120 mm): tieplate_small:3 ↔ M3_Lock_Nut(Thin_Nut):31
- Cylindrical:27: M3 X 10mm Screw:36 ↔ M3_Lock_Nut(Thin_Nut):30
- Cylindrical:28: M3 X 10mm Screw:33 ↔ M3_Lock_Nut(Thin_Nut):34
- Cylindrical:29: M3 X 10mm Screw:30 ↔ M3_Lock_Nut(Thin_Nut):37
- Cylindrical:30: M3 X 10mm Screw:35 ↔ M3_Lock_Nut(Thin_Nut):33
- Cylindrical:31: M3 X 10mm Screw:27 ↔ M3_Lock_Nut(Thin_Nut):36
- Cylindrical:32: M3 X 10mm Screw:32 ↔ M3_Lock_Nut(Thin_Nut):31
- Cylindrical:33: M3 X 10mm Screw:25 ↔ M3_Lock_Nut(Thin_Nut):32
- Cylindrical:34: M3 X 10mm Screw:28 ↔ M3_Lock_Nut(Thin_Nut):28
- Cylindrical:35: M3 X 10mm Screw:34 ↔ M3_Lock_Nut(Thin_Nut):35
- Cylindrical:38: M3 X 10mm Screw:31 ↔ M3_Lock_Nut(Thin_Nut):27
- Cylindrical:36: M3 X 10mm Screw:29 ↔ M3_Lock_Nut(Thin_Nut):29
- Cylindrical:37: M3 X 10mm Screw:26 ↔ M3_Lock_Nut(Thin_Nut):26
- Mate:74: tieplate_small:2 ↔ M3 X 10mm Screw:25
- Mate:75: tieplate_small:2 ↔ M3 X 10mm Screw:28
- Mate:76: tieplate_small:2 ↔ M3 X 10mm Screw:34
- Mate:77: tieplate_small:2 ↔ M3 X 10mm Screw:31
- Mate:78: tieplate_small:2 ↔ M3 X 10mm Screw:29
- Mate:79: tieplate_small:2 ↔ M3 X 10mm Screw:26
- Mate:80: tieplate_small:3 ↔ M3 X 10mm Screw:35
- Mate:81: tieplate_small:3 ↔ M3 X 10mm Screw:30
- Mate:82: tieplate_small:3 ↔ M3 X 10mm Screw:27
- Mate:83: tieplate_small:3 ↔ M3 X 10mm Screw:33
- Mate:84: tieplate_small:3 ↔ M3 X 10mm Screw:36
- Mate:85: tieplate_small:3 ↔ M3 X 10mm Screw:32
- Slider:37 [TranslationJoint]: makerbeam600mm:3 ↔ M3_Lock_Nut(Thin_Nut):39
- Slider:38 [TranslationJoint]: makerbeam600mm:3 ↔ M3_Lock_Nut(Thin_Nut):40
- Slider:39 [TranslationJoint]: makerbeam600mm:2 ↔ M3_Lock_Nut(Thin_Nut):42
- Slider:40 [TranslationJoint]: makerbeam600mm:2 ↔ M3_Lock_Nut(Thin_Nut):41
- Mate:86 (-10.5 mm): tieplate_big:1 ↔ M3_Lock_Nut(Thin_Nut):39
- Mate:87 (-60.5 mm): tieplate_big:1 ↔ M3_Lock_Nut(Thin_Nut):40
- Mate:88 (-10.5 mm): tieplate_big:1 ↔ M3_Lock_Nut(Thin_Nut):41
- Mate:89 (-60.5 mm): tieplate_big:1 ↔ M3_Lock_Nut(Thin_Nut):42
- Cylindrical:39: M3_Lock_Nut(Thin_Nut):40 ↔ M3 X 10mm Screw:37
- Cylindrical:42: M3_Lock_Nut(Thin_Nut):39 ↔ M3 X 10mm Screw:38
- Cylindrical:40: M3_Lock_Nut(Thin_Nut):42 ↔ M3 X 10mm Screw:39
- Cylindrical:41: M3_Lock_Nut(Thin_Nut):41 ↔ M3 X 10mm Screw:40
- Mate:90: tieplate_big:1 ↔ M3 X 10mm Screw:38
- Mate:91: tieplate_big:1 ↔ M3 X 10mm Screw:37
- Mate:92: tieplate_big:1 ↔ M3 X 10mm Screw:39
- Mate:93: tieplate_big:1 ↔ M3 X 10mm Screw:40
- Mate:94: tieplate_small:6 ↔ makerbeam876mm:2
- Mate:95: makerbeam600mm:2 ↔ makerbeam876mm:2
- Mate:96: tieplate_small:6 ↔ makerbeam876mm:1
- Flush:54: tieplate_small:6 ↔ makerbeam876mm:1
- Mate:97: makerbeam600mm:3 ↔ makerbeam876mm:4
- Mate:98: tieplate_small:7 ↔ makerbeam876mm:4
- Mate:99: tieplate_small:7 ↔ makerbeam876mm:3
- Flush:55: tieplate_small:7 ↔ makerbeam876mm:3
- Flush:56 (-52.0465 mm): tieplate_small:7 ↔ makerbeam876mm:3
- Flush:57 (-52.0465 mm): tieplate_small:6 ↔ makerbeam876mm:1
- Flush:58 (-52.0465 mm): tieplate_small:7 ↔ makerbeam876mm:4
- Flush:59 (-52.0465 mm): tieplate_small:6 ↔ makerbeam876mm:2
- Slider:41 [TranslationJoint]: makerbeam876mm:4 ↔ M3_Lock_Nut(Thin_Nut):45
- Slider:42 [TranslationJoint]: makerbeam876mm:4 ↔ M3_Lock_Nut(Thin_Nut):44